# Autodesk Inventor assembly: calebs minimal extruder
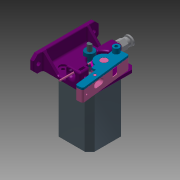
[picture p0: Inventor's stored thumbnail of the model, 180x180]
Saved by Autodesk Inventor 2014 (Build 180170000, 170)
## iProperties
Created: 2014-11-01
Part Number: calebs minimal extruder
Document SubType Name: Assembly
Designer: caleb
Author: caleb
## Documents named in this file (12)
- C:\cygwin\home\caleb\caleb-typea-settings\designs\bowden-extruder\calebs minimal extruder.iam
- C:\cygwin\home\caleb\caleb-typea-settings\designs\bowden-extruder\extruder base.ipt
- C:\cygwin\home\caleb\caleb-typea-settings\designs\bowden-extruder\nema 17 motor.ipt
- C:\cygwin\home\caleb\caleb-typea-settings\designs\bowden-extruder\drive gear.ipt
- C:\cygwin\home\caleb\caleb-typea-settings\designs\bowden-extruder\filament.ipt
- C:\cygwin\home\caleb\caleb-typea-settings\designs\bowden-extruder\bearing.ipt
- C:\cygwin\home\caleb\caleb-typea-settings\designs\bowden-extruder\tensioner 1.ipt
- C:\cygwin\home\caleb\caleb-typea-settings\designs\bowden-extruder\tensioner 2.ipt
- C:\cygwin\home\caleb\caleb-typea-settings\designs\bowden-extruder\tensioner washer.ipt
- C:\cygwin\home\caleb\caleb-typea-settings\designs\bowden-extruder\tension release wedge.ipt
- C:\cygwin\home\caleb\caleb-typea-settings\designs\bowden-extruder\Part1.ipt
- C:\cygwin\home\caleb\caleb-typea-settings\designs\bowden-extruder\push-fitting.ipt
## Components (11 placed, 11 different names)
1. extruder base:1 — Mate:8, Mate:9, Mate:11
2. nema 17 motor:1
3. drive gear:1
4. filament:1 — Mate:10
5. bearing:1 — Mate:1, Mate:2, Mate:4
6. tensioner 1:1 — Mate:1, Mate:2, Mate:3, Mate:6, Mate:7, Mate:9, Mate:12
7. tensioner 2:1 — Mate:6, Mate:7, Mate:8, Mate:12
8. tensioner washer:1 — Mate:3, Mate:4
9. tension release wedge:1
10. Part1:1
11. push-fitting:1 — Mate:10, Mate:11
## Relationships (11: Mate 11)
- Mate:1: bearing:1 ↔ tensioner 1:1
- Mate:2: bearing:1 ↔ tensioner 1:1
- Mate:3: tensioner 1:1 ↔ tensioner washer:1
- Mate:4: bearing:1 ↔ tensioner washer:1
- Mate:6: tensioner 1:1 ↔ tensioner 2:1
- Mate:7: tensioner 1:1 ↔ tensioner 2:1
- Mate:8: extruder base:1 ↔ tensioner 2:1
- Mate:9 (0.1 mm): extruder base:1 ↔ tensioner 1:1
- Mate:10: filament:1 ↔ push-fitting:1
- Mate:11 (1.385 mm): extruder base:1 ↔ push-fitting:1
- Mate:12: tensioner 1:1 ↔ tensioner 2:1
